# Autodesk Inventor assembly: A_Aft
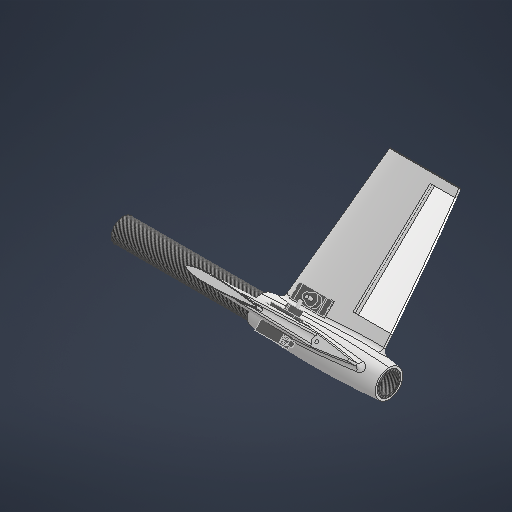
[picture p0: Inventor's stored thumbnail of the model, 512x512]
Saved by Autodesk Inventor 2026 (Build 300175000, 175)
## iProperties
Created: 2025-09-10
Part Number: A_Aft
Document SubType Name: Assembly
Designer: FAL
Author: FAL
## Documents named in this file (5)
- C:\Users\FAL\Projekte\Git\AIRBERT\CAD\Aft\A_Aft.iam
- C:\Users\FAL\Projekte\Git\AIRBERT\CAD\Aft\P_aft_V.ipt
- C:\Users\FAL\Projekte\Git\AIRBERT\CAD\Aft\P_aft_V_rudder.ipt
- C:\Users\FAL\Projekte\Git\AIRBERT\CAD\Aft\P_Carbon_Pipe_Back.ipt
- C:\Users\FAL\Projekte\Git\AIRBERT\CAD\Electronic\P_Servo_27x12.ipt
## Components (5 placed, 4 different names)
1. P_aft_V:1 — Fluchtend:1, Fluchtend:2, Fluchtend:3, Fluchtend:10, Passend:1, Passend:2, Passend:3, Passend:4, Passend:5, Passend:6
2. P_aft_V_rudder:1 — Fluchtend:4, Fluchtend:5, Fluchtend:6
3. P_Carbon_Pipe_Back:1 — Fluchtend:8, Fluchtend:9, Fluchtend:10
4. P_Servo_27x12:1 — Passend:1, Passend:3, Passend:4
5. P_Servo_27x12:2 — Passend:2, Passend:5, Passend:6
## Relationships (15: Flush 9, Mate 6)
- Fluchtend:1 [Flush]: P_aft_V:1
- Fluchtend:2 [Flush]: P_aft_V:1
- Fluchtend:3 [Flush]: P_aft_V:1
- Fluchtend:4 [Flush]: P_aft_V_rudder:1
- Fluchtend:5 [Flush]: P_aft_V_rudder:1
- Fluchtend:6 [Flush]: P_aft_V_rudder:1
- Fluchtend:8 [Flush]: P_Carbon_Pipe_Back:1
- Fluchtend:9 [Flush]: P_Carbon_Pipe_Back:1
- Fluchtend:10 [Flush]: P_aft_V:1 ↔ P_Carbon_Pipe_Back:1
- Passend:1 [Mate]: P_aft_V:1 ↔ P_Servo_27x12:1
- Passend:2 [Mate]: P_aft_V:1 ↔ P_Servo_27x12:2
- Passend:3 [Mate]: P_aft_V:1 ↔ P_Servo_27x12:1
- Passend:4 [Mate]: P_aft_V:1 ↔ P_Servo_27x12:1
- Passend:5 [Mate]: P_aft_V:1 ↔ P_Servo_27x12:2
- Passend:6 [Mate]: P_aft_V:1 ↔ P_Servo_27x12:2
